# Autodesk Inventor assembly: Korpus_Einbau
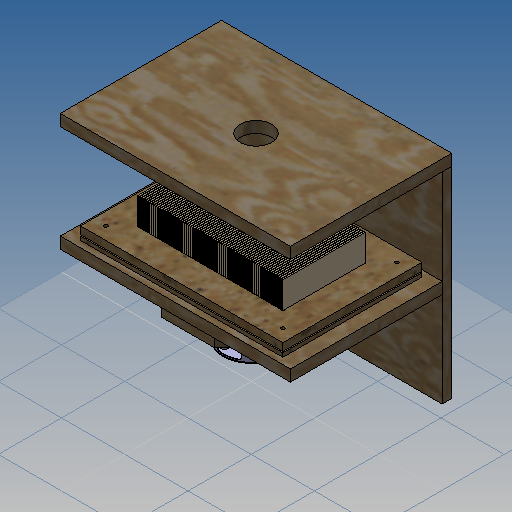
[picture p0: Inventor's stored thumbnail of the model, 512x512]
Saved by Autodesk Inventor 2019 (Build 230136000, 136)
## iProperties
Created: 2020-08-04
Part Number: Korpus_Einbau
Material: Generisch
Document SubType Name: Assembly
Designer: Stefan
Mass: 7450 g
Surface Area: 21226.5 cm^2
Volume: 7373.14 cm^3
Density: 1.01042 g/cm^3
Author: Stefan
## Documents named in this file (10)
- C:\Users\User\OneDrive\Dokumente\Inventor\Absauganlage\Korpus_Einbau.iam
- C:\Users\User\OneDrive\Dokumente\Inventor\Absauganlage\Korpus_Einbau_Basis.ipt
- C:\Users\User\OneDrive\Dokumente\Inventor\Absauganlage\Korpus_Einbau_Rücken.ipt
- C:\Users\User\OneDrive\Dokumente\Inventor\Absauganlage\Korpus_Einbau_Deckel.ipt
- C:\Users\User\OneDrive\Dokumente\Inventor\Absauganlage\Korpus_Motor_18mm.ipt
- C:\Users\User\OneDrive\Dokumente\Inventor\Absauganlage\Korpus_Motor_15mm.ipt
- C:\Users\User\OneDrive\Dokumente\Inventor\Absauganlage\Import\Vacuum_Motor\ASSEMBELY\Motor1.iam
- C:\Users\User\OneDrive\Dokumente\Inventor\Absauganlage\Flachfaltenfilter_Rahmen.ipt
- C:\Users\User\OneDrive\Dokumente\Inventor\Absauganlage\Flachfaltenfilte_240x140.ipt
- C:\Users\User\OneDrive\Dokumente\Inventor\Absauganlage\Flachfaltenfilter_Basis.ipt
## Components (9 placed, 9 different names)
1. Korpus_Einbau_Basis:1 — Passend:1, Fluchtend:1, Passend:3, Passend:6, Passend:7, Winkel:1, Passend:8, Passend:16, Passend:17, Passend:18, Passend:19, Passend:20
2. Korpus_Einbau_Rücken:1 — Passend:1, Fluchtend:1, Passend:2, Fluchtend:2, Fluchtend:3
3. Korpus_Einbau_Deckel:1 — Passend:2, Fluchtend:2, Fluchtend:3, Passend:3
4. Korpus_Motor_18mm:1 — Passend:4, Passend:5, Fluchtend:4, Passend:6, Passend:7, Winkel:1
5. Korpus_Motor_15mm:1 — Passend:4, Passend:5, Fluchtend:4, Passend:9
6. Motor1:1 [sub-assembly] — Passend:8, Passend:9
7. Flachfaltenfilter_Rahmen:1 — Passend:13, Passend:14, Passend:15, Passend:16, Passend:17
8. Flachfaltenfilte_240x140:1 — Passend:13, Passend:14, Passend:15, Passend:21
9. Flachfaltenfilter_Basis:1 — Passend:18, Passend:19, Passend:20, Passend:21
## Relationships (23: Mate 18, Flush 4, Angle 1)
- Passend:1 [Mate]: Korpus_Einbau_Basis:1 ↔ Korpus_Einbau_Rücken:1
- Fluchtend:1 [Flush]: Korpus_Einbau_Basis:1 ↔ Korpus_Einbau_Rücken:1
- Passend:2 [Mate]: Korpus_Einbau_Rücken:1 ↔ Korpus_Einbau_Deckel:1
- Fluchtend:2 [Flush]: Korpus_Einbau_Rücken:1 ↔ Korpus_Einbau_Deckel:1
- Fluchtend:3 [Flush]: Korpus_Einbau_Rücken:1 ↔ Korpus_Einbau_Deckel:1
- Passend:3 [Mate] (150 mm): Korpus_Einbau_Basis:1 ↔ Korpus_Einbau_Deckel:1
- Passend:4 [Mate]: Korpus_Motor_18mm:1 ↔ Korpus_Motor_15mm:1
- Passend:5 [Mate]: Korpus_Motor_18mm:1 ↔ Korpus_Motor_15mm:1
- Fluchtend:4 [Flush]: Korpus_Motor_18mm:1 ↔ Korpus_Motor_15mm:1
- Passend:6 [Mate]: Korpus_Einbau_Basis:1 ↔ Korpus_Motor_18mm:1
- Passend:7 [Mate]: Korpus_Einbau_Basis:1 ↔ Korpus_Motor_18mm:1
- Winkel:1 [Angle] (0 deg): Korpus_Einbau_Basis:1 ↔ Korpus_Motor_18mm:1
- Passend:8 [Mate]: Korpus_Einbau_Basis:1 ↔ Motor1:1
- Passend:9 [Mate]: Korpus_Motor_15mm:1 ↔ Motor1:1
- Passend:13 [Mate]: Flachfaltenfilter_Rahmen:1 ↔ Flachfaltenfilte_240x140:1
- Passend:14 [Mate]: Flachfaltenfilter_Rahmen:1 ↔ Flachfaltenfilte_240x140:1
- Passend:15 [Mate]: Flachfaltenfilter_Rahmen:1 ↔ Flachfaltenfilte_240x140:1
- Passend:16 [Mate]: Korpus_Einbau_Basis:1 ↔ Flachfaltenfilter_Rahmen:1
- Passend:17 [Mate]: Korpus_Einbau_Basis:1 ↔ Flachfaltenfilter_Rahmen:1
- Passend:18 [Mate]: Korpus_Einbau_Basis:1 ↔ Flachfaltenfilter_Basis:1
- Passend:19 [Mate]: Korpus_Einbau_Basis:1 ↔ Flachfaltenfilter_Basis:1
- Passend:20 [Mate]: Korpus_Einbau_Basis:1 ↔ Flachfaltenfilter_Basis:1
- Passend:21 [Mate]: Flachfaltenfilte_240x140:1 ↔ Flachfaltenfilter_Basis:1
